# Autodesk Inventor assembly: ASY ДМФ 010 крышка
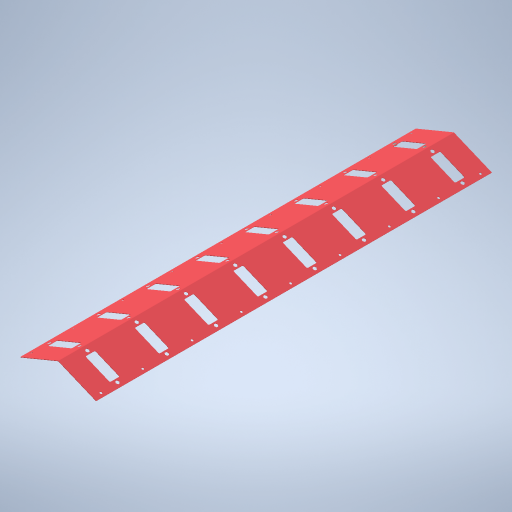
[picture p0: Inventor's stored thumbnail of the model, 512x512]
Saved by Autodesk Inventor 2024.2 (Build 282272000, 272)
## iProperties
Created: 2024-04-30
Part Number: ASY ДМФ 010 крышка
Document SubType Name: Assembly
Designer: admin
Author: admin
## Documents named in this file (5)
- C:\Users\admin\YandexDisk-badmisterfox\домашниий пк\Inventor\DMF-Disk-Micro-Filter\ASY ДМФ 010 крышка.iam
- C:\Users\admin\YandexDisk-badmisterfox\домашниий пк\Inventor\DMF-Disk-Micro-Filter\ДМФ 01 11 Барабан Лист крышка.ipt
- C:\Users\admin\YandexDisk-badmisterfox\домашниий пк\Inventor\DMF-Disk-Micro-Filter\ДМФ 01 12 Барабан усилитель.ipt
- C:\Users\admin\YandexDisk-badmisterfox\домашниий пк\Inventor\DMF-Disk-Micro-Filter\ContentCenter\en-US\ISO 4032(1)\ISO 4032 - M10DIN EN.ipt
- C:\Users\admin\YandexDisk-badmisterfox\домашниий пк\Inventor\DMF-Disk-Micro-Filter\Knife.ipt
## Components (20 placed, 4 different names)
1. ДМФ 01 11 Барабан Лист крышка:1 — Mate:1, Mate:2, Flush:1, Mate:4, Mate:5, Mate:6, Mate:7, Flush:5, Flush:6
2. DIN EN 24032 M10:1 — Mate:4, Mate:5, Flush:6
3. DIN EN 24032 M10:2 — Mate:6, Mate:7, Flush:5
4. Knife:1 — Flush:7
5. ДМФ 01 12 Барабан усилитель:2 — Rigid:1
6. ДМФ 01 12 Барабан усилитель:1 — Mate:1, Mate:2, Rigid:1
7. ДМФ 01 12 Барабан усилитель:3
8. ДМФ 01 12 Барабан усилитель:4
9. ДМФ 01 12 Барабан усилитель:5
10. ДМФ 01 12 Барабан усилитель:6
11. ДМФ 01 12 Барабан усилитель:7
12. ДМФ 01 12 Барабан усилитель:8
13. ДМФ 01 12 Барабан усилитель:9
14. ДМФ 01 12 Барабан усилитель:10
15. ДМФ 01 12 Барабан усилитель:11
16. ДМФ 01 12 Барабан усилитель:12
17. ДМФ 01 12 Барабан усилитель:13
18. ДМФ 01 12 Барабан усилитель:14
19. ДМФ 01 12 Барабан усилитель:15 — Flush:1
20. ДМФ 01 12 Барабан усилитель:16
## Component patterns: (8 elements, first: ДМФ 01 12 Барабан усилитель:2 + ДМФ 01 12 Барабан усилитель:1)
## Relationships (11: Mate 6, Flush 4, WeldJoint 1)
- Mate:1: ДМФ 01 11 Барабан Лист крышка:1 ↔ ДМФ 01 12 Барабан усилитель:1
- Mate:2: ДМФ 01 11 Барабан Лист крышка:1 ↔ ДМФ 01 12 Барабан усилитель:1
- Rigid:1 [WeldJoint] (108 mm): ДМФ 01 12 Барабан усилитель:2 ↔ ДМФ 01 12 Барабан усилитель:1
- Flush:1 (29 mm): ДМФ 01 11 Барабан Лист крышка:1 ↔ ДМФ 01 12 Барабан усилитель:15
- Mate:4: ДМФ 01 11 Барабан Лист крышка:1 ↔ DIN EN 24032 M10:1
- Mate:5: ДМФ 01 11 Барабан Лист крышка:1 ↔ DIN EN 24032 M10:1
- Mate:6: ДМФ 01 11 Барабан Лист крышка:1 ↔ DIN EN 24032 M10:2
- Mate:7: ДМФ 01 11 Барабан Лист крышка:1 ↔ DIN EN 24032 M10:2
- Flush:5: ДМФ 01 11 Барабан Лист крышка:1 ↔ DIN EN 24032 M10:2
- Flush:6: ДМФ 01 11 Барабан Лист крышка:1 ↔ DIN EN 24032 M10:1
- Flush:7: Knife:1
